# Autodesk Inventor assembly: robot
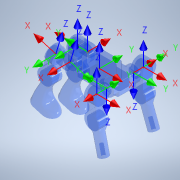
[picture p0: Inventor's stored thumbnail of the model, 180x180]
Saved by Autodesk Inventor 2020.2 (Build 242310000, 310)
## iProperties
Created: 2021-01-29
Part Number: robot
Document SubType Name: Assembly
Designer: DELL
Author: DELL
## Documents named in this file (8)
- D:\repo\experimental_flexipod\mesh\v7.0\robot.iam
- D:\repo\experimental_flexipod\mesh\v7.0\body.ipt
- D:\repo\experimental_flexipod\mesh\v7.0\hip.ipt
- D:\repo\experimental_flexipod\mesh\v7.0\thigh.ipt
- D:\repo\experimental_flexipod\mesh\v7.0\shank_2.ipt
- D:\repo\experimental_flexipod\mesh\v7.0\hip_back.ipt
- D:\repo\experimental_flexipod\mesh\v7.0\hip_back_mirror.ipt
- D:\repo\experimental_flexipod\mesh\v7.0\shank_front.ipt
## Components (13 placed, 7 different names)
1. body:1 — Flush:1, Flush:2, Flush:3, Mate:1, Mate:2, Mate:3, Mate:4, Angle:4, Angle:5, Angle:6, Angle:7, Angle:15, Angle:16, Angle:17, Mate:31, Mate:32, Mate:35, Mate:36, Angle:18
2. hip:1 — Mate:3, Mate:4, Mate:10, Mate:14, Angle:5
3. hip:2 — Mate:1, Mate:2, Mate:9, Flush:4, Angle:7
4. thigh:1 — Mate:9, Flush:4, Angle:17, Mate:44, Flush:43
5. thigh:2 — Mate:10, Mate:14, Angle:6, Mate:43, Flush:42
6. thigh:3 — Angle:16, Mate:33, Mate:34, Mate:42, Flush:41
7. thigh:4 — Angle:4, Angle:15, Flush:38, Mate:37, Angle:18, Mate:41, Flush:40
8. hip_back:1 — Mate:31, Mate:32, Mate:33, Mate:34
9. hip_back_mirror:1 — Mate:35, Mate:36, Flush:38, Mate:37
10. shank_2:3 — Mate:41, Flush:40
11. shank_2:4 — Mate:42, Flush:41
12. shank_front:1 — Mate:43, Flush:42
13. shank_front:2 — Mate:44, Flush:43
## Relationships (35: Mate 18, Flush 9, Angle 8)
- Flush:1: body:1
- Flush:2: body:1
- Flush:3: body:1
- Mate:1: body:1 ↔ hip:2
- Mate:2: body:1 ↔ hip:2
- Mate:3: body:1 ↔ hip:1
- Mate:4: body:1 ↔ hip:1
- Mate:9: hip:2 ↔ thigh:1
- Mate:10: hip:1 ↔ thigh:2
- Flush:4: hip:2 ↔ thigh:1
- Mate:14: hip:1 ↔ thigh:2
- Angle:4 (0 deg): body:1 ↔ thigh:4
- Angle:5 (0 deg): body:1 ↔ hip:1
- Angle:6 (0 deg): body:1 ↔ thigh:2
- Angle:7 (0 deg): body:1 ↔ hip:2
- Angle:15 (0 deg): body:1 ↔ thigh:4
- Angle:16 (0 deg): body:1 ↔ thigh:3
- Angle:17 (0 deg): body:1 ↔ thigh:1
- Mate:31: body:1 ↔ hip_back:1
- Mate:32: body:1 ↔ hip_back:1
- Mate:33: thigh:3 ↔ hip_back:1
- Mate:34: thigh:3 ↔ hip_back:1
- Mate:35: body:1 ↔ hip_back_mirror:1
- Mate:36: body:1 ↔ hip_back_mirror:1
- Flush:38: thigh:4 ↔ hip_back_mirror:1
- Mate:37: thigh:4 ↔ hip_back_mirror:1
- Angle:18 (0 deg): body:1 ↔ thigh:4
- Mate:41: thigh:4 ↔ shank_2:3
- Flush:40: thigh:4 ↔ shank_2:3
- Mate:42: thigh:3 ↔ shank_2:4
- Flush:41: thigh:3 ↔ shank_2:4
- Mate:43: thigh:2 ↔ shank_front:1
- Mate:44: thigh:1 ↔ shank_front:2
- Flush:42: thigh:2 ↔ shank_front:1
- Flush:43: thigh:1 ↔ shank_front:2
